# Autodesk Inventor assembly: Assembly1
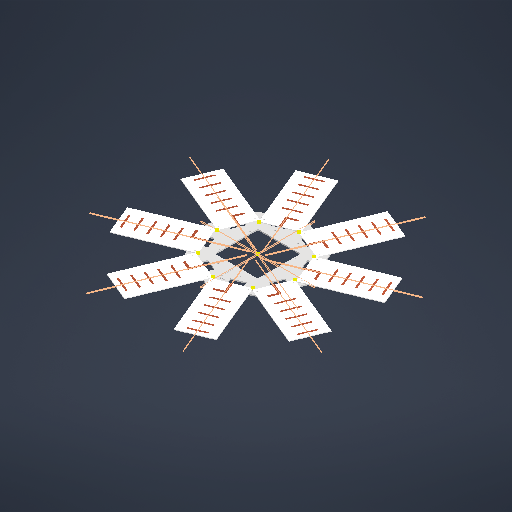
[picture p0: Inventor's stored thumbnail of the model, 512x512]
Saved by Autodesk Inventor 2026.1 (Build 301233020, 233B)
## iProperties
Created: 2026-05-13
Part Number: Assembly1
Document SubType Name: Assembly
Designer: Mikke
Author: Mikke
## Documents named in this file (3)
- C:\Users\Mikke\OneDrive - Aalborg Universitet\ESD 610 - General\Inventor\Blomsten\Assembly1.iam
- C:\Users\Mikke\OneDrive - Aalborg Universitet\ESD 610 - General\Inventor\Cover_image\Bund.ipt
- C:\Users\Mikke\OneDrive - Aalborg Universitet\ESD 610 - General\Inventor\Cover_image\Antenna.ipt
## Components (9 placed, 2 different names)
1. Bund:1 — Mate:1, Mate:2, Mate:3
2. Antenna:1 — Mate:1, Mate:2, Mate:3
3. Antenna:2
4. Antenna:3
5. Antenna:4
6. Antenna:5
7. Antenna:6
8. Antenna:7
9. Antenna:8
## Component patterns: (8 elements, first: Antenna:1)
## Relationships (3: Mate 3)
- Mate:1: Bund:1 ↔ Antenna:1
- Mate:2: Bund:1 ↔ Antenna:1
- Mate:3: Bund:1 ↔ Antenna:1
